# Autodesk Inventor assembly: A2017_T4_08
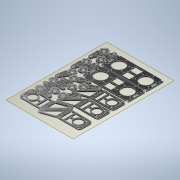
[picture p0: Inventor's stored thumbnail of the model, 180x180]
Saved by Autodesk Inventor 2022 (Build 260153000, 153)
## iProperties
Created: 2022-09-28
Part Number: A2017_T4_08
Document SubType Name: Assembly
Designer: Masato
Author: Masato
## Documents named in this file (5)
- C:\Users\MasatoKubotera\Documents\Inventor\SUSTAINA-OP\Cam\A2017_T4\A2017_T4_08.iam
- C:\Users\MasatoKubotera\Documents\Inventor\SUSTAINA-OP\Cam\DisposableBoard.ipt
- C:\Users\MasatoKubotera\Documents\Inventor\SUSTAINA-OP\LowerBody\Ankle\Ankle_side_pitch_frame.ipt
- C:\Users\MasatoKubotera\Documents\Inventor\SUSTAINA-OP\UpperBody\Trunk\Trunk_shoulder_frame.ipt
- C:\Users\MasatoKubotera\Documents\Inventor\SUSTAINA-OP\UpperBody\Trunk\Trunk_waisit_frame.ipt
## Components (19 placed, 4 different names)
1. DisposableBoard:1 — フラッシュ:1, フラッシュ:2, フラッシュ:3, フラッシュ:4, フラッシュ:5, 正接:1, フラッシュ:6
2. Ankle_side_pitch_frame:1 — メイト:2, 正接:2, メイト:10, メイト:11
3. Ankle_side_pitch_frame:2 — メイト:3, メイト:11, 正接:3, 正接:4, メイト:22
4. Trunk_shoulder_frame:1 — メイト:4, 正接:1, フラッシュ:6, メイト:7, フラッシュ:7, フラッシュ:8
5. Trunk_shoulder_frame:2 — メイト:5, フラッシュ:7, メイト:8, フラッシュ:9, メイト:20
6. Ankle_side_pitch_frame:7 — メイト:14, メイト:22, メイト:23, 正接:5, 正接:27
7. Ankle_side_pitch_frame:9 — メイト:12, メイト:20, 正接:4, 正接:20
8. Trunk_shoulder_frame:4 — メイト:17, 正接:20, フラッシュ:9, 正接:6, メイト:25
9. Ankle_side_pitch_frame:14 — メイト:15, メイト:23, 正接:6, 正接:21, 正接:24
10. Trunk_shoulder_frame:5 — メイト:6, フラッシュ:5, メイト:7, メイト:8, 正接:2, メイト:10, 正接:3, 正接:5, フラッシュ:10, 正接:26
11. Ankle_side_pitch_frame:15 — メイト:24, メイト:25, 正接:21, 正接:22, 正接:25
12. Ankle_side_pitch_frame:16 — メイト:26, 正接:23, 正接:24, 正接:25, 正接:28
13. Ankle_side_pitch_frame:17 — メイト:27, 正接:26, 正接:27, 正接:28, 正接:29, 正接:30
14. Trunk_waisit_frame:2 — メイト:9, フラッシュ:8, 正接:22, 正接:23, メイト:31
15. Trunk_waisit_frame:3
16. Ankle_side_pitch_frame:18 — フラッシュ:10, メイト:28, メイト:29, 正接:29
17. Ankle_side_pitch_frame:19 — メイト:28, メイト:30, メイト:31, 正接:30
18. Ankle_side_pitch_frame:20
19. Ankle_side_pitch_frame:21
## Component patterns: (2 elements, first: Trunk_waisit_frame:2), (2 elements, first: Ankle_side_pitch_frame:18 + Ankle_side_pitch_frame:19)
## Relationships (52: Mate 25, Tangent 17, Flush 10)
- フラッシュ:1 [Flush]: DisposableBoard:1
- フラッシュ:2 [Flush]: DisposableBoard:1
- フラッシュ:3 [Flush]: DisposableBoard:1
- フラッシュ:4 [Flush]: DisposableBoard:1
- メイト:2 [Mate]: Ankle_side_pitch_frame:1
- メイト:3 [Mate]: Ankle_side_pitch_frame:2
- メイト:4 [Mate]: Trunk_shoulder_frame:1
- メイト:5 [Mate]: Trunk_shoulder_frame:2
- メイト:6 [Mate]: Trunk_shoulder_frame:5
- フラッシュ:5 [Flush] (2 mm): DisposableBoard:1 ↔ Trunk_shoulder_frame:5
- 正接:1 [Tangent] (2 mm): DisposableBoard:1 ↔ Trunk_shoulder_frame:1
- フラッシュ:6 [Flush] (2 mm): DisposableBoard:1 ↔ Trunk_shoulder_frame:1
- メイト:7 [Mate] (2.1 mm): Trunk_shoulder_frame:1 ↔ Trunk_shoulder_frame:5
- フラッシュ:7 [Flush]: Trunk_shoulder_frame:1 ↔ Trunk_shoulder_frame:2
- メイト:8 [Mate] (2.1 mm): Trunk_shoulder_frame:2 ↔ Trunk_shoulder_frame:5
- メイト:9 [Mate]: Trunk_waisit_frame:2
- フラッシュ:8 [Flush]: Trunk_shoulder_frame:1 ↔ Trunk_waisit_frame:2
- 正接:2 [Tangent]: Ankle_side_pitch_frame:1 ↔ Trunk_shoulder_frame:5
- メイト:10 [Mate] (2.1 mm): Ankle_side_pitch_frame:1 ↔ Trunk_shoulder_frame:5
- メイト:11 [Mate] (2.1 mm): Ankle_side_pitch_frame:1 ↔ Ankle_side_pitch_frame:2
- メイト:12 [Mate]: Ankle_side_pitch_frame:9
- メイト:14 [Mate]: Ankle_side_pitch_frame:7
- メイト:15 [Mate]: Ankle_side_pitch_frame:14
- メイト:17 [Mate]: Trunk_shoulder_frame:4
- 正接:20 [Tangent] (2.1 mm): Ankle_side_pitch_frame:9 ↔ Trunk_shoulder_frame:4
- フラッシュ:9 [Flush]: Trunk_shoulder_frame:2 ↔ Trunk_shoulder_frame:4
- メイト:20 [Mate] (2.1 mm): Trunk_shoulder_frame:2 ↔ Ankle_side_pitch_frame:9
- 正接:22 [Tangent] (2.1 mm): Ankle_side_pitch_frame:15 ↔ Trunk_waisit_frame:2
- 正接:3 [Tangent]: Ankle_side_pitch_frame:2 ↔ Trunk_shoulder_frame:5
- 正接:4 [Tangent] (2.1 mm): Ankle_side_pitch_frame:2 ↔ Ankle_side_pitch_frame:9
- メイト:22 [Mate] (2.1 mm): Ankle_side_pitch_frame:2 ↔ Ankle_side_pitch_frame:7
- メイト:23 [Mate] (2.1 mm): Ankle_side_pitch_frame:7 ↔ Ankle_side_pitch_frame:14
- 正接:5 [Tangent]: Ankle_side_pitch_frame:7 ↔ Trunk_shoulder_frame:5
- 正接:6 [Tangent] (2.1 mm): Trunk_shoulder_frame:4 ↔ Ankle_side_pitch_frame:14
- メイト:24 [Mate]: Ankle_side_pitch_frame:15
- メイト:25 [Mate] (2.1 mm): Trunk_shoulder_frame:4 ↔ Ankle_side_pitch_frame:15
- 正接:21 [Tangent] (2.1 mm): Ankle_side_pitch_frame:14 ↔ Ankle_side_pitch_frame:15
- メイト:26 [Mate]: Ankle_side_pitch_frame:16
- 正接:23 [Tangent] (2.1 mm): Ankle_side_pitch_frame:16 ↔ Trunk_waisit_frame:2
- 正接:24 [Tangent] (2.1 mm): Ankle_side_pitch_frame:14 ↔ Ankle_side_pitch_frame:16
- 正接:25 [Tangent] (2.1 mm): Ankle_side_pitch_frame:15 ↔ Ankle_side_pitch_frame:16
- メイト:27 [Mate]: Ankle_side_pitch_frame:17
- フラッシュ:10 [Flush]: Trunk_shoulder_frame:5 ↔ Ankle_side_pitch_frame:18
- メイト:28 [Mate] (2.1 mm): Ankle_side_pitch_frame:18 ↔ Ankle_side_pitch_frame:19
- 正接:26 [Tangent]: Trunk_shoulder_frame:5 ↔ Ankle_side_pitch_frame:17
- メイト:29 [Mate]: Ankle_side_pitch_frame:18
- メイト:30 [Mate]: Ankle_side_pitch_frame:19
- メイト:31 [Mate] (2.1 mm): Trunk_waisit_frame:2 ↔ Ankle_side_pitch_frame:19
- 正接:27 [Tangent] (2.1 mm): Ankle_side_pitch_frame:7 ↔ Ankle_side_pitch_frame:17
- 正接:28 [Tangent] (2.1 mm): Ankle_side_pitch_frame:16 ↔ Ankle_side_pitch_frame:17
- 正接:29 [Tangent] (2.1 mm): Ankle_side_pitch_frame:17 ↔ Ankle_side_pitch_frame:18
- 正接:30 [Tangent] (2.1 mm): Ankle_side_pitch_frame:17 ↔ Ankle_side_pitch_frame:19
